# Autodesk Inventor assembly: RT_FRM_A_003_FrameV2
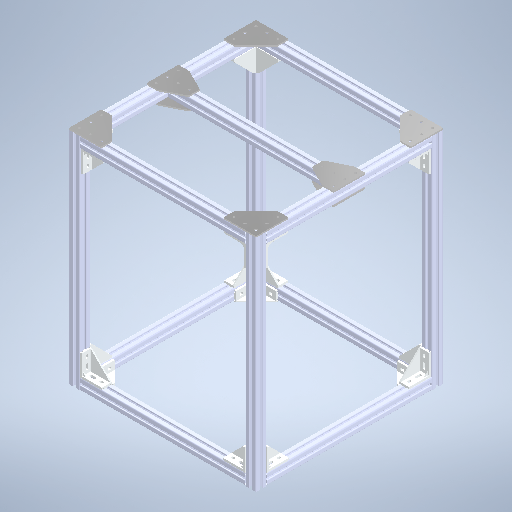
[picture p0: Inventor's stored thumbnail of the model, 512x512]
Saved by Autodesk Inventor 2025.3 (Build 293356000, 356)
## iProperties
Created: 2026-05-11
Part Number: RT_FRM_A_003_FrameV2
Document SubType Name: Assembly
Designer: louis
Mass: 15556.7 g
Surface Area: 56486.4 cm^2
Volume: 5761.74 cm^3
Density: 2.7 g/cm^3
Author: louis
## Documents named in this file (12)
- C:\Users\louis\OneDrive\Desktop\R_Trident\02_CAD\04_Subassemblies\RT_FRM_A_003_FrameV2.iam
- C:\Users\louis\OneDrive\Desktop\R_Trident\02_CAD\01_Standard_Parts\Aluminium_Extrusions\4040x800_3619_20251007144627_4040.ipt
- C:\Users\louis\OneDrive\Desktop\R_Trident\02_CAD\01_Standard_Parts\Aluminium_Extrusions\4040x600_3619_20251007144627_4040.ipt
- C:\Users\louis\OneDrive\Desktop\R_Trident\02_CAD\01_Standard_Parts\3532_20210408113519_4080L + cover\3532_20210408113519_4080L + cover.iam
- C:\Users\louis\OneDrive\Desktop\R_Trident\02_CAD\01_Standard_Parts\Connection_plate_L_120x120.ipt
- C:\Users\louis\OneDrive\Desktop\R_Trident\02_CAD\01_Standard_Parts\Connection_plate_T_120x120.ipt
- C:\Users\louis\OneDrive\Desktop\R_Trident\02_CAD\04_Subassemblies\RT_FRM_A_003_FrameV2\AIP\FEA\fg1z6mt7k.fins
- C:\Users\louis\OneDrive\Desktop\R_Trident\02_CAD\04_Subassemblies\RT_FRM_A_003_FrameV2\AIP\FEA\fg1z6mt7k.fsat
- C:\Users\louis\OneDrive\Desktop\R_Trident\02_CAD\04_Subassemblies\RT_FRM_A_003_FrameV2\AIP\FEA\fg1z6mt7k.ftes
- C:\Users\louis\OneDrive\Desktop\R_Trident\02_CAD\04_Subassemblies\RT_FRM_A_003_FrameV2\AIP\FEA\fg1z6mt7k.fwiz
- C:\Users\louis\OneDrive\Desktop\R_Trident\02_CAD\04_Subassemblies\RT_FRM_A_003_FrameV2\AIP\FEA\fg1z6mtb4.fmsh
- C:\Users\louis\OneDrive\Desktop\R_Trident\02_CAD\04_Subassemblies\RT_FRM_A_003_FrameV2\AIP\FEA\fg1z6mtb5.fres
## Components (41 placed, 5 different names)
1. 4040x800_3619_20251007144627_4040:1 — Flush:2, Mate:2, Mate:4, Flush:6, Flush:12, Flush:13, Mate:11, Mate:13, Flush:19, Flush:24, Flush:25, Mate:24, Flush:37, Flush:39, Mate:28, Mate:54, Flush:58, Mate:56
2. 4040x800_3619_20251007144627_4040:2 — Flush:1, Flush:2, Flush:3, Mate:5, Mate:8, Flush:10, Flush:11, Mate:12, Flush:22, Flush:23, Mate:34, Mate:36, Mate:45, Mate:48
3. 4040x800_3619_20251007144627_4040:3 — Flush:3, Mate:3, Mate:6, Flush:5, Flush:14, Flush:15, Mate:10, Flush:18, Flush:20, Flush:26, Flush:27, Mate:17, Flush:34, Mate:20, Mate:58, Mate:59
4. 4040x800_3619_20251007144627_4040:4 — Flush:1, Mate:7, Mate:9, Flush:4, Flush:7, Flush:8, Flush:9, Flush:16, Flush:17, Flush:21, Flush:28, Mate:41, Mate:44, Mate:50, Mate:51
5. 4040x600_3619_20251007144627_4040:1 — Mate:2, Mate:3, Flush:5, Flush:13, Flush:14, Symmetry:1, Mate:29, Flush:42, Flush:45, Mate:53, Mate:60, Flush:61
6. 4040x600_3619_20251007144627_4040:2 — Mate:4, Mate:5, Flush:6, Flush:11, Flush:12, Mate:15, Flush:30, Symmetry:2, Symmetry:3, Mate:30, Mate:31, Flush:43, Flush:44, Mate:46, Flush:54, Mate:55, Flush:59, Mate:63, Flush:64, Flush:65
7. 4040x600_3619_20251007144627_4040:3 — Mate:6, Mate:7, Flush:4, Flush:9, Flush:15, Mate:14, Flush:29, Symmetry:3, Mate:32, Flush:40, Flush:41, Mate:52, Flush:57, Mate:57, Flush:60, Mate:61, Flush:62, Flush:63
8. 4040x600_3619_20251007144627_4040:4 — Mate:8, Mate:9, Flush:7, Flush:8, Flush:10, Symmetry:1, Flush:46, Flush:47, Mate:47, Flush:55, Mate:49, Flush:56
9. 4040x600_3619_20251007144627_4040:5 — Mate:10, Flush:16, Flush:20, Flush:27, Flush:28, Flush:35, Mate:19, Flush:36, Mate:22, Flush:51, Mate:39, Flush:52, Mate:42
10. 4040x600_3619_20251007144627_4040:6 — Mate:11, Flush:19, Flush:23, Flush:24, Symmetry:2, Flush:38, Mate:26, Mate:27, Flush:49, Mate:35, Flush:50, Mate:37
11. 4040x600_3619_20251007144627_4040:7 — Mate:13, Flush:18, Flush:25, Flush:26, Mate:18, Mate:21, Mate:23, Mate:25
12. 4040x600_3619_20251007144627_4040:8 — Mate:12, Flush:17, Flush:21, Flush:22, Flush:48, Mate:33, Mate:38, Mate:40, Mate:43, Flush:53
13. 4040x600_3619_20251007144627_4040:9 — Mate:14, Mate:15, Flush:29, Flush:30, Flush:31, Mate:62, Mate:64
14. 3532_20210408113519_4080L + cover:1 [sub-assembly] — Mate:17, Flush:34, Mate:18
15. 3532_20210408113519_4080L + cover:2 [sub-assembly] — Flush:35, Mate:19, Mate:20
16. 3532_20210408113519_4080L + cover:3 [sub-assembly] — Mate:21, Flush:36, Mate:22
17. 3532_20210408113519_4080L + cover:4 [sub-assembly] — Mate:23, Mate:24, Flush:37
18. 3532_20210408113519_4080L + cover:5 [sub-assembly] — Flush:39, Mate:27, Mate:28
19. 3532_20210408113519_4080L + cover:6 [sub-assembly] — Mate:25, Flush:38, Mate:26
20. Connection_plate_L_120x120:1 — Mate:29, Flush:41, Flush:45
21. Connection_plate_L_120x120:2 — Mate:32, Flush:40, Flush:46
22. Connection_plate_L_120x120:3 — Mate:30, Flush:42, Flush:44
23. Connection_plate_L_120x120:4 — Mate:31, Flush:43, Flush:47
24. 3532_20210408113519_4080L + cover:7 [sub-assembly] — Flush:49, Mate:35, Mate:36
25. 3532_20210408113519_4080L + cover:8 [sub-assembly] — Flush:50, Mate:37, Mate:38
26. 3532_20210408113519_4080L + cover:9 [sub-assembly] — Flush:48, Mate:33, Mate:34
27. 3532_20210408113519_4080L + cover:10 [sub-assembly] — Flush:51, Mate:39, Mate:40
28. 3532_20210408113519_4080L + cover:11 [sub-assembly] — Mate:43, Mate:44, Flush:53
29. 3532_20210408113519_4080L + cover:12 [sub-assembly] — Flush:52, Mate:41, Mate:42
30. 3532_20210408113519_4080L + cover:13 [sub-assembly] — Mate:45, Mate:46, Flush:54
31. 3532_20210408113519_4080L + cover:14 [sub-assembly] — Mate:47, Mate:48, Flush:55
32. 3532_20210408113519_4080L + cover:15 [sub-assembly] — Mate:51, Mate:52, Flush:57
33. 3532_20210408113519_4080L + cover:16 [sub-assembly] — Mate:49, Mate:50, Flush:56
34. 3532_20210408113519_4080L + cover:17 [sub-assembly] — Mate:53, Mate:54, Flush:58
35. 3532_20210408113519_4080L + cover:18 [sub-assembly] — Mate:55, Mate:56, Flush:59
36. 3532_20210408113519_4080L + cover:19 [sub-assembly] — Mate:57, Mate:58, Flush:60
37. 3532_20210408113519_4080L + cover:20 [sub-assembly] — Mate:59, Mate:60, Flush:61
38. Connection_plate_T_120x120:1 — Mate:61, Flush:62, Mate:65
39. Connection_plate_T_120x120:2 — Mate:62, Flush:63, Flush:66
40. Connection_plate_T_120x120:3 — Mate:63, Flush:64, Flush:67
41. Connection_plate_T_120x120:4 — Mate:64, Flush:65, Flush:68
## Relationships (135: Flush 68, Mate 64, Symmetry 3)
- Flush:1: 4040x800_3619_20251007144627_4040:2 ↔ 4040x800_3619_20251007144627_4040:4
- Flush:2: 4040x800_3619_20251007144627_4040:1 ↔ 4040x800_3619_20251007144627_4040:2
- Flush:3: 4040x800_3619_20251007144627_4040:2 ↔ 4040x800_3619_20251007144627_4040:3
- Mate:2: 4040x800_3619_20251007144627_4040:1 ↔ 4040x600_3619_20251007144627_4040:1
- Mate:3: 4040x800_3619_20251007144627_4040:3 ↔ 4040x600_3619_20251007144627_4040:1
- Mate:4: 4040x800_3619_20251007144627_4040:1 ↔ 4040x600_3619_20251007144627_4040:2
- Mate:5: 4040x800_3619_20251007144627_4040:2 ↔ 4040x600_3619_20251007144627_4040:2
- Mate:6: 4040x800_3619_20251007144627_4040:3 ↔ 4040x600_3619_20251007144627_4040:3
- Mate:7: 4040x800_3619_20251007144627_4040:4 ↔ 4040x600_3619_20251007144627_4040:3
- Mate:8: 4040x800_3619_20251007144627_4040:2 ↔ 4040x600_3619_20251007144627_4040:4
- Mate:9: 4040x800_3619_20251007144627_4040:4 ↔ 4040x600_3619_20251007144627_4040:4
- Flush:4: 4040x800_3619_20251007144627_4040:4 ↔ 4040x600_3619_20251007144627_4040:3
- Flush:5: 4040x800_3619_20251007144627_4040:3 ↔ 4040x600_3619_20251007144627_4040:1
- Flush:6: 4040x800_3619_20251007144627_4040:1 ↔ 4040x600_3619_20251007144627_4040:2
- Flush:7: 4040x800_3619_20251007144627_4040:4 ↔ 4040x600_3619_20251007144627_4040:4
- Flush:8: 4040x800_3619_20251007144627_4040:4 ↔ 4040x600_3619_20251007144627_4040:4
- Flush:9: 4040x800_3619_20251007144627_4040:4 ↔ 4040x600_3619_20251007144627_4040:3
- Flush:10: 4040x800_3619_20251007144627_4040:2 ↔ 4040x600_3619_20251007144627_4040:4
- Flush:11: 4040x800_3619_20251007144627_4040:2 ↔ 4040x600_3619_20251007144627_4040:2
- Flush:12: 4040x800_3619_20251007144627_4040:1 ↔ 4040x600_3619_20251007144627_4040:2
- Flush:13: 4040x800_3619_20251007144627_4040:1 ↔ 4040x600_3619_20251007144627_4040:1
- Flush:14: 4040x800_3619_20251007144627_4040:3 ↔ 4040x600_3619_20251007144627_4040:1
- Flush:15: 4040x800_3619_20251007144627_4040:3 ↔ 4040x600_3619_20251007144627_4040:3
- Mate:10: 4040x800_3619_20251007144627_4040:3 ↔ 4040x600_3619_20251007144627_4040:5
- Mate:11: 4040x800_3619_20251007144627_4040:1 ↔ 4040x600_3619_20251007144627_4040:6
- Mate:12: 4040x800_3619_20251007144627_4040:2 ↔ 4040x600_3619_20251007144627_4040:8
- Mate:13: 4040x800_3619_20251007144627_4040:1 ↔ 4040x600_3619_20251007144627_4040:7
- Flush:16: 4040x800_3619_20251007144627_4040:4 ↔ 4040x600_3619_20251007144627_4040:5
- Flush:17: 4040x800_3619_20251007144627_4040:4 ↔ 4040x600_3619_20251007144627_4040:8
- Flush:18: 4040x800_3619_20251007144627_4040:3 ↔ 4040x600_3619_20251007144627_4040:7
- Flush:19: 4040x800_3619_20251007144627_4040:1 ↔ 4040x600_3619_20251007144627_4040:6
- Flush:20: 4040x800_3619_20251007144627_4040:3 ↔ 4040x600_3619_20251007144627_4040:5
- Flush:21: 4040x800_3619_20251007144627_4040:4 ↔ 4040x600_3619_20251007144627_4040:8
- Flush:22: 4040x800_3619_20251007144627_4040:2 ↔ 4040x600_3619_20251007144627_4040:8
- Flush:23: 4040x800_3619_20251007144627_4040:2 ↔ 4040x600_3619_20251007144627_4040:6
- Flush:24: 4040x800_3619_20251007144627_4040:1 ↔ 4040x600_3619_20251007144627_4040:6
- Flush:25: 4040x800_3619_20251007144627_4040:1 ↔ 4040x600_3619_20251007144627_4040:7
- Flush:26: 4040x800_3619_20251007144627_4040:3 ↔ 4040x600_3619_20251007144627_4040:7
- Flush:27: 4040x800_3619_20251007144627_4040:3 ↔ 4040x600_3619_20251007144627_4040:5
- Flush:28: 4040x800_3619_20251007144627_4040:4 ↔ 4040x600_3619_20251007144627_4040:5
- Mate:14: 4040x600_3619_20251007144627_4040:3 ↔ 4040x600_3619_20251007144627_4040:9
- Mate:15: 4040x600_3619_20251007144627_4040:2 ↔ 4040x600_3619_20251007144627_4040:9
- Flush:29: 4040x600_3619_20251007144627_4040:3 ↔ 4040x600_3619_20251007144627_4040:9
- Flush:30: 4040x600_3619_20251007144627_4040:2 ↔ 4040x600_3619_20251007144627_4040:9
- Symmetry:1: 4040x600_3619_20251007144627_4040:1 ↔ 4040x600_3619_20251007144627_4040:4
- Symmetry:2: 4040x600_3619_20251007144627_4040:2 ↔ 4040x600_3619_20251007144627_4040:6
- Flush:31: 4040x600_3619_20251007144627_4040:9
- Flush:32
- Flush:33
- Symmetry:3: 4040x600_3619_20251007144627_4040:2 ↔ 4040x600_3619_20251007144627_4040:3
- Mate:16
- Mate:17: 4040x800_3619_20251007144627_4040:3 ↔ 3532_20210408113519_4080L + cover:1
- Flush:34: 4040x800_3619_20251007144627_4040:3 ↔ 3532_20210408113519_4080L + cover:1
- Mate:18: 4040x600_3619_20251007144627_4040:7 ↔ 3532_20210408113519_4080L + cover:1
- Flush:35: 4040x600_3619_20251007144627_4040:5 ↔ 3532_20210408113519_4080L + cover:2
- Mate:19: 4040x600_3619_20251007144627_4040:5 ↔ 3532_20210408113519_4080L + cover:2
- Mate:20: 4040x800_3619_20251007144627_4040:3 ↔ 3532_20210408113519_4080L + cover:2
- Mate:21: 4040x600_3619_20251007144627_4040:7 ↔ 3532_20210408113519_4080L + cover:3
- Flush:36: 4040x600_3619_20251007144627_4040:5 ↔ 3532_20210408113519_4080L + cover:3
- Mate:22: 4040x600_3619_20251007144627_4040:5 ↔ 3532_20210408113519_4080L + cover:3
- Mate:23: 4040x600_3619_20251007144627_4040:7 ↔ 3532_20210408113519_4080L + cover:4
- Mate:24: 4040x800_3619_20251007144627_4040:1 ↔ 3532_20210408113519_4080L + cover:4
- Flush:37: 4040x800_3619_20251007144627_4040:1 ↔ 3532_20210408113519_4080L + cover:4
- Mate:25: 4040x600_3619_20251007144627_4040:7 ↔ 3532_20210408113519_4080L + cover:6
- Flush:38: 4040x600_3619_20251007144627_4040:6 ↔ 3532_20210408113519_4080L + cover:6
- Mate:26: 4040x600_3619_20251007144627_4040:6 ↔ 3532_20210408113519_4080L + cover:6
- Flush:39: 4040x800_3619_20251007144627_4040:1 ↔ 3532_20210408113519_4080L + cover:5
- Mate:27: 4040x600_3619_20251007144627_4040:6 ↔ 3532_20210408113519_4080L + cover:5
- Mate:28: 4040x800_3619_20251007144627_4040:1 ↔ 3532_20210408113519_4080L + cover:5
- Mate:29: 4040x600_3619_20251007144627_4040:1 ↔ Connection_plate_L_120x120:1
- Mate:30: 4040x600_3619_20251007144627_4040:2 ↔ Connection_plate_L_120x120:3
- Mate:31: 4040x600_3619_20251007144627_4040:2 ↔ Connection_plate_L_120x120:4
- Mate:32: 4040x600_3619_20251007144627_4040:3 ↔ Connection_plate_L_120x120:2
- Flush:40: 4040x600_3619_20251007144627_4040:3 ↔ Connection_plate_L_120x120:2
- Flush:41: 4040x600_3619_20251007144627_4040:3 ↔ Connection_plate_L_120x120:1
- Flush:42: 4040x600_3619_20251007144627_4040:1 ↔ Connection_plate_L_120x120:3
- Flush:43: 4040x600_3619_20251007144627_4040:2 ↔ Connection_plate_L_120x120:4
- Flush:44: 4040x600_3619_20251007144627_4040:2 ↔ Connection_plate_L_120x120:3
- Flush:45: 4040x600_3619_20251007144627_4040:1 ↔ Connection_plate_L_120x120:1
- Flush:46: 4040x600_3619_20251007144627_4040:4 ↔ Connection_plate_L_120x120:2
- Flush:47: 4040x600_3619_20251007144627_4040:4 ↔ Connection_plate_L_120x120:4
- Flush:48: 4040x600_3619_20251007144627_4040:8 ↔ 3532_20210408113519_4080L + cover:9
- Mate:33: 4040x600_3619_20251007144627_4040:8 ↔ 3532_20210408113519_4080L + cover:9
- Mate:34: 4040x800_3619_20251007144627_4040:2 ↔ 3532_20210408113519_4080L + cover:9
- Flush:49: 4040x600_3619_20251007144627_4040:6 ↔ 3532_20210408113519_4080L + cover:7
- Mate:35: 4040x600_3619_20251007144627_4040:6 ↔ 3532_20210408113519_4080L + cover:7
- Mate:36: 4040x800_3619_20251007144627_4040:2 ↔ 3532_20210408113519_4080L + cover:7
- Flush:50: 4040x600_3619_20251007144627_4040:6 ↔ 3532_20210408113519_4080L + cover:8
- Mate:37: 4040x600_3619_20251007144627_4040:6 ↔ 3532_20210408113519_4080L + cover:8
- Mate:38: 4040x600_3619_20251007144627_4040:8 ↔ 3532_20210408113519_4080L + cover:8
- Flush:51: 4040x600_3619_20251007144627_4040:5 ↔ 3532_20210408113519_4080L + cover:10
- Mate:39: 4040x600_3619_20251007144627_4040:5 ↔ 3532_20210408113519_4080L + cover:10
- Mate:40: 4040x600_3619_20251007144627_4040:8 ↔ 3532_20210408113519_4080L + cover:10
- Flush:52: 4040x600_3619_20251007144627_4040:5 ↔ 3532_20210408113519_4080L + cover:12
- Mate:41: 4040x800_3619_20251007144627_4040:4 ↔ 3532_20210408113519_4080L + cover:12
- Mate:42: 4040x600_3619_20251007144627_4040:5 ↔ 3532_20210408113519_4080L + cover:12
- Mate:43: 4040x600_3619_20251007144627_4040:8 ↔ 3532_20210408113519_4080L + cover:11
- Mate:44: 4040x800_3619_20251007144627_4040:4 ↔ 3532_20210408113519_4080L + cover:11
- Flush:53: 4040x600_3619_20251007144627_4040:8 ↔ 3532_20210408113519_4080L + cover:11
- Mate:45: 4040x800_3619_20251007144627_4040:2 ↔ 3532_20210408113519_4080L + cover:13
- Mate:46: 4040x600_3619_20251007144627_4040:2 ↔ 3532_20210408113519_4080L + cover:13
- Flush:54: 4040x600_3619_20251007144627_4040:2 ↔ 3532_20210408113519_4080L + cover:13
- Mate:47: 4040x600_3619_20251007144627_4040:4 ↔ 3532_20210408113519_4080L + cover:14
- Mate:48: 4040x800_3619_20251007144627_4040:2 ↔ 3532_20210408113519_4080L + cover:14
- Flush:55: 4040x600_3619_20251007144627_4040:4 ↔ 3532_20210408113519_4080L + cover:14
- Mate:49: 4040x600_3619_20251007144627_4040:4 ↔ 3532_20210408113519_4080L + cover:16
- Mate:50: 4040x800_3619_20251007144627_4040:4 ↔ 3532_20210408113519_4080L + cover:16
- Flush:56: 4040x600_3619_20251007144627_4040:4 ↔ 3532_20210408113519_4080L + cover:16
- Mate:51: 4040x800_3619_20251007144627_4040:4 ↔ 3532_20210408113519_4080L + cover:15
- Mate:52: 4040x600_3619_20251007144627_4040:3 ↔ 3532_20210408113519_4080L + cover:15
- Flush:57: 4040x600_3619_20251007144627_4040:3 ↔ 3532_20210408113519_4080L + cover:15
- Mate:53: 4040x600_3619_20251007144627_4040:1 ↔ 3532_20210408113519_4080L + cover:17
- Mate:54: 4040x800_3619_20251007144627_4040:1 ↔ 3532_20210408113519_4080L + cover:17
- Flush:58: 4040x800_3619_20251007144627_4040:1 ↔ 3532_20210408113519_4080L + cover:17
- Mate:55: 4040x600_3619_20251007144627_4040:2 ↔ 3532_20210408113519_4080L + cover:18
- Mate:56: 4040x800_3619_20251007144627_4040:1 ↔ 3532_20210408113519_4080L + cover:18
- Flush:59: 4040x600_3619_20251007144627_4040:2 ↔ 3532_20210408113519_4080L + cover:18
- Mate:57: 4040x600_3619_20251007144627_4040:3 ↔ 3532_20210408113519_4080L + cover:19
- Mate:58: 4040x800_3619_20251007144627_4040:3 ↔ 3532_20210408113519_4080L + cover:19
- Flush:60: 4040x600_3619_20251007144627_4040:3 ↔ 3532_20210408113519_4080L + cover:19
- Mate:59: 4040x800_3619_20251007144627_4040:3 ↔ 3532_20210408113519_4080L + cover:20
- Mate:60: 4040x600_3619_20251007144627_4040:1 ↔ 3532_20210408113519_4080L + cover:20
- Flush:61: 4040x600_3619_20251007144627_4040:1 ↔ 3532_20210408113519_4080L + cover:20
- Mate:61: 4040x600_3619_20251007144627_4040:3 ↔ Connection_plate_T_120x120:1
- Flush:62: 4040x600_3619_20251007144627_4040:3 ↔ Connection_plate_T_120x120:1
- Mate:62: 4040x600_3619_20251007144627_4040:9 ↔ Connection_plate_T_120x120:2
- Flush:63: 4040x600_3619_20251007144627_4040:3 ↔ Connection_plate_T_120x120:2
- Mate:63: 4040x600_3619_20251007144627_4040:2 ↔ Connection_plate_T_120x120:3
- Flush:64: 4040x600_3619_20251007144627_4040:2 ↔ Connection_plate_T_120x120:3
- Mate:64: 4040x600_3619_20251007144627_4040:9 ↔ Connection_plate_T_120x120:4
- Flush:65: 4040x600_3619_20251007144627_4040:2 ↔ Connection_plate_T_120x120:4
- Mate:65: Connection_plate_T_120x120:1
- Flush:66: Connection_plate_T_120x120:2
- Flush:67: Connection_plate_T_120x120:3
- Flush:68: Connection_plate_T_120x120:4
## Named parameters: sa_0 = 10000, sa_1 = 20000
note: some values were not read from the file. Shown as the stored number, unit unknown: "sa_0", "sa_1".
